# Autodesk Inventor assembly: 2018_radiator_assembly2018 sidepontoon assenbly2
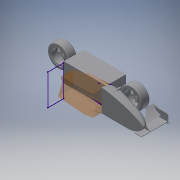
[picture p0: Inventor's stored thumbnail of the model, 180x180]
Saved by Autodesk Inventor 2018 (Build 220112000, 112)
## iProperties
Company: none
Created: 2018-02-24
Part Number: 2018_radiator_assembly2018 sidepontoon assenbly2
Material: 一般
Description: CATIA V5 STEP Exchange
Document SubType Name: Assembly
Designer: KITformula
Authority: none
Title: Z:\各班フォルダ\2018\ボディ\カウル\AeroCAD2018\CAD\Inventor\Aero Parts\Side Pontoon\2018 sidepontoon assenbly2.stp
Author: none
Sending System: CATIA V5 STEP AP203
Preprocessor: CATIA Version 5 Release 17 (IN-10)
## Documents named in this file (8)
- Z:\各班フォルダ\2018\ボディ\カウル\AeroCAD2018\CAD\Inventor\Aero Parts\Side Pontoon\2018_radiator_assembly2018 sidepontoon assenbly2.iam
- Z:\各班フォルダ\2018\ボディ\カウル\AeroCAD2018\CAD\Inventor\Aero Parts\Side Pontoon\2018_radiator_assembly2radiator 2018.ipt
- Z:\各班フォルダ\2018\ボディ\カウル\AeroCAD2018\CAD\Inventor\Aero Parts\Side Pontoon\2018_radiator_assembly2AssyTsutsui2018.iam
- Z:\各班フォルダ\2018\ボディ\カウル\AeroCAD2018\CAD\Inventor\Aero Parts\Side Pontoon\2018_radiator_assembly2SidePanel_Upper1.ipt
- Z:\各班フォルダ\2018\ボディ\カウル\AeroCAD2018\CAD\Inventor\Aero Parts\Side Pontoon\2018_radiator_assembly2aaa.ipt
- Z:\各班フォルダ\2018\ボディ\カウル\AeroCAD2018\CAD\Inventor\Aero Parts\Side Pontoon\2018_radiator_assembly2F-wing.iam
- Z:\各班フォルダ\2018\ボディ\カウル\AeroCAD2018\CAD\Inventor\Aero Parts\Side Pontoon\2018_radiator_assembly2underpanel middle.ipt
- Z:\各班フォルダ\2018\ボディ\カウル\AeroCAD2018\CAD\Inventor\Aero Parts\Side Pontoon\Side pontoon2.ipt
## Components (7 placed, 7 different names)
1. radiator 2018.1
2. AssyTsutsui2018.1 [sub-assembly]
3. Part127.1
4. 2018Frontnose
5. F-wing.1 [sub-assembly]
6. underpanel middle.1
7. Side pontoon2:1 — メイト:1
## Relationships (1: Mate 1)
- メイト:1 [Mate]: Side pontoon2:1
